# Autodesk Inventor assembly: couple extension arm motor middle + pulleys
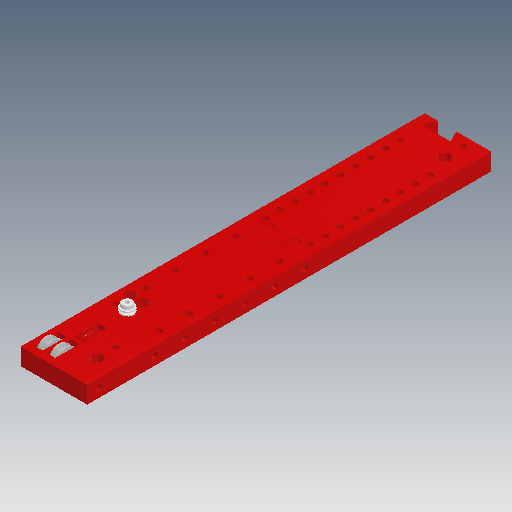
[picture p0: Inventor's stored thumbnail of the model, 512x512]
Saved by Autodesk Inventor 2020 (Build 240168000, 168)
## iProperties
Created: 2019-12-16
Part Number: couple extension arm motor middle + pulleys
Document SubType Name: Assembly
Designer: ball
Author: ball
## Documents named in this file (6)
- C:\FTC\FTC8863CAD\2019 Robot\Delivery\extension arm\couple extension arm motor top + pulleys.iam
- C:\FTC\FTC8863CAD\2019 Robot\Delivery\extension arm\Coupler extension arm motor.ipt
- C:\FTC\FTC8863CAD\2019 Robot\Delivery\plastic pulley deep u.ipt
- C:\FTC\FTC8863CAD\RevRobotics\REV-41-1368 pulley.ipt
- C:\FTC\FTC8863CAD\StepLibraries\Screws\M3 x 8 SOCKET HEAD CAP SCREW.ipt
- C:\FTC\FTC8863CAD\StepLibraries\Washers\M3 FLAT WASHER.ipt
## Components (7 placed, 5 different names)
1. Coupler extension arm motor:1 — Mate:1, Mate:2, Mate:3, Mate:4, Mate:5, Mate:6, Mate:7, Mate:13
2. plastic pulley deep u:1 — Mate:3, Mate:4
3. REV-41-1368 pulley:1 — Mate:1, Mate:2
4. REV-41-1368 pulley:2 — Mate:5, Mate:6
5. M3 x 8 SOCKET HEAD CAP SCREW:1 — Mate:11, Mate:12
6. M3 FLAT WASHER:1 — Mate:9, Mate:10, Mate:11, Mate:12
7. M3 FLAT WASHER:2 — Mate:7, Mate:9, Mate:10, Mate:13
## Relationships (12: Mate 12)
- Mate:1: Coupler extension arm motor:1 ↔ REV-41-1368 pulley:1
- Mate:2: Coupler extension arm motor:1 ↔ REV-41-1368 pulley:1
- Mate:3: Coupler extension arm motor:1 ↔ plastic pulley deep u:1
- Mate:4: Coupler extension arm motor:1 ↔ plastic pulley deep u:1
- Mate:5: Coupler extension arm motor:1 ↔ REV-41-1368 pulley:2
- Mate:6: Coupler extension arm motor:1 ↔ REV-41-1368 pulley:2
- Mate:7: Coupler extension arm motor:1 ↔ M3 FLAT WASHER:2
- Mate:9 (1 mm): M3 FLAT WASHER:1 ↔ M3 FLAT WASHER:2
- Mate:10: M3 FLAT WASHER:1 ↔ M3 FLAT WASHER:2
- Mate:11: M3 x 8 SOCKET HEAD CAP SCREW:1 ↔ M3 FLAT WASHER:1
- Mate:12: M3 x 8 SOCKET HEAD CAP SCREW:1 ↔ M3 FLAT WASHER:1
- Mate:13: Coupler extension arm motor:1 ↔ M3 FLAT WASHER:2
